# Autodesk Inventor assembly: Assembly1
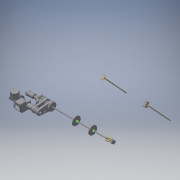
[picture p0: Inventor's stored thumbnail of the model, 180x180]
Saved by Autodesk Inventor 2019 (Build 230136000, 136)
## iProperties
Created: 2019-04-27
Part Number: Assembly1
Document SubType Name: Assembly
Designer: isadmin
Author: isadmin
## Documents named in this file (17)
- C:\Users\isadmin\Documents\Inventor\IS_01\Assembly1.iam
- C:\Users\isadmin\Documents\Inventor\IS_01\670000.ipt
- C:\Users\isadmin\Documents\Inventor\IS_01\CF Insert Flange Support 01.ipt
- C:\Users\isadmin\Documents\Inventor\IS_01\MCF275-FlgMplxr-Cr1A5_(53-321020-A).ipt
- C:\Users\isadmin\Documents\Inventor\IS_01\665501.ipt
- C:\Users\isadmin\Documents\Inventor\IS_01\Rod Central.ipt
- C:\Users\isadmin\Documents\Inventor\IS_01\block.ipt
- C:\Users\isadmin\Documents\Inventor\IS_01\Shield_1.ipt
- C:\Users\isadmin\Documents\Inventor\IS_01\Shield_3.ipt
- C:\Users\isadmin\Documents\Inventor\IS_01\Shutter.ipt
- C:\Users\isadmin\Documents\Inventor\IS_01\ceramic washer.ipt
- C:\Users\isadmin\Documents\Inventor\IS_01\Shielding.ipt
- C:\Users\isadmin\Documents\Inventor\IS_01\alumina_standoff_LSP_ASO00110.ipt
- C:\Users\isadmin\Documents\Inventor\IS_01\Bullet_v5_SiliconeSample.ipt
- C:\Users\isadmin\Documents\Inventor\IS_01\Bullet_v5_SiliconeSample_TopPart.ipt
- C:\Users\isadmin\Documents\Inventor\IS_01\Part8.ipt
- C:\Users\isadmin\Documents\Inventor\IS_01\Part9.ipt
## Components (43 placed, 16 different names)
1. 670000:1 — Insert:1, Insert:4
2. CF Insert Flange Support:1 — Insert:3
3. MCF275-FlgMplxr-Cr1A5_(53-321020-A):1 — Insert:1, Insert:2
4. 665501:1 — Insert:2, Insert:3
5. Rod Central:1 — Insert:4, Insert:5, Insert:7, Insert:8
6. block:1 — Insert:6
7. Shield_1:1 — Mate:32
8. Shield_3:1 — Insert:5
9. Shutter:1
10. ceramic washer:1
11. ceramic washer:2
12. ceramic washer:3
13. ceramic washer:4
14. Shielding:1
15. ceramic washer:5
16. ceramic washer:6
17. ceramic washer:7
18. ceramic washer:8
19. alumina_standoff_LSP_ASO00110:1
20. alumina_standoff_LSP_ASO00110:2
21. alumina_standoff_LSP_ASO00110:3 — Mate:32
22. alumina_standoff_LSP_ASO00110:4
23. Bullet_v5_SiliconeSample:1 — Insert:6
24. Bullet_v5_SiliconeSample_TopPart:1
25. Part8:1 — Insert:7, Insert:9
26. Part8:2 — Insert:8, Insert:10
27. Part9:1 — Insert:9
28. Part9:2 — Insert:10
29. Shield_1:2 — Insert:12, Insert:13
30. block:2 — Insert:12, Insert:13
31. Shutter:2
32. ceramic washer:9
33. ceramic washer:10
34. ceramic washer:11
35. ceramic washer:12
36. Shielding:2
37. ceramic washer:13
38. ceramic washer:14
39. ceramic washer:15
40. ceramic washer:16
41. Bullet_v5_SiliconeSample:2
42. Bullet_v5_SiliconeSample_TopPart:2
43. Shield_1:3
## Relationships (75: Mate 56, Insert 13, Flush 6)
- Insert:1 (-0.254 mm): 670000:1 ↔ MCF275-FlgMplxr-Cr1A5_(53-321020-A):1
- Insert:2 (0.254 mm): MCF275-FlgMplxr-Cr1A5_(53-321020-A):1 ↔ 665501:1
- Insert:3 (0.254 mm): CF Insert Flange Support:1 ↔ 665501:1
- Insert:4: 670000:1 ↔ Rod Central:1
- [Mate]: block:1 ↔ Shield_1:1
- [Flush]: block:1 ↔ Shield_1:1
- [Flush]: block:1 ↔ Shield_1:1
- [Mate]: block:1 ↔ Shutter:1
- [Mate]: block:1 ↔ Shutter:1
- [Mate]: block:1 ↔ Shutter:1
- [Mate]: block:1 ↔ ceramic washer:2
- [Mate]: block:1 ↔ ceramic washer:2
- [Mate]: block:1 ↔ ceramic washer:1
- [Mate]: block:1 ↔ ceramic washer:1
- [Mate]: block:1 ↔ ceramic washer:4
- [Mate]: block:1 ↔ ceramic washer:4
- [Mate]: block:1 ↔ ceramic washer:3
- [Mate]: block:1 ↔ ceramic washer:3
- [Mate]: ceramic washer:1 ↔ Shielding:1
- [Flush]: block:1 ↔ Shielding:1
- [Flush]: block:1 ↔ Shielding:1
- [Mate]: block:1 ↔ ceramic washer:5
- [Mate]: block:1 ↔ ceramic washer:5
- [Mate]: block:1 ↔ ceramic washer:6
- [Mate]: block:1 ↔ ceramic washer:6
- [Mate]: block:1 ↔ ceramic washer:7
- [Mate]: block:1 ↔ ceramic washer:7
- [Mate]: block:1 ↔ ceramic washer:8
- [Mate]: block:1 ↔ ceramic washer:8
- [Mate]: Shield_1:1 ↔ alumina_standoff_LSP_ASO00110:3
- [Mate]: Shield_1:1 ↔ alumina_standoff_LSP_ASO00110:2
- [Mate]: Shield_1:1 ↔ alumina_standoff_LSP_ASO00110:2
- [Mate]: Shield_1:1 ↔ alumina_standoff_LSP_ASO00110:4
- [Mate]: Shield_1:1 ↔ alumina_standoff_LSP_ASO00110:4
- [Mate]: Shield_1:1 ↔ alumina_standoff_LSP_ASO00110:1
- [Mate]: Shield_1:1 ↔ alumina_standoff_LSP_ASO00110:1
- [Mate]: Shield_3:1 ↔ alumina_standoff_LSP_ASO00110:3
- [Mate]: Shield_3:1 ↔ alumina_standoff_LSP_ASO00110:2
- [Mate]: Shield_3:1 ↔ alumina_standoff_LSP_ASO00110:2
- Mate:32: Shield_1:1 ↔ alumina_standoff_LSP_ASO00110:3
- Insert:5: Rod Central:1 ↔ Shield_3:1
- [Mate] (0.0254 mm): Bullet_v5_SiliconeSample:1 ↔ Bullet_v5_SiliconeSample_TopPart:1
- [Mate]: Bullet_v5_SiliconeSample:1 ↔ Bullet_v5_SiliconeSample_TopPart:1
- Insert:6: block:1 ↔ Bullet_v5_SiliconeSample:1
- Insert:7 (-304.8 mm): Rod Central:1 ↔ Part8:1
- Insert:8 (-152.4 mm): Rod Central:1 ↔ Part8:2
- Insert:9 (-12.7 mm): Part8:1 ↔ Part9:1
- Insert:10 (-12.7 mm): Part8:2 ↔ Part9:2
- [Mate]: block:2 ↔ Shutter:2
- [Mate]: block:2 ↔ Shutter:2
- [Mate]: block:2 ↔ Shutter:2
- [Mate]: block:2 ↔ ceramic washer:10
- [Mate]: block:2 ↔ ceramic washer:10
- [Mate]: block:2 ↔ ceramic washer:9
- [Mate]: block:2 ↔ ceramic washer:9
- [Mate]: block:2 ↔ ceramic washer:12
- [Mate]: block:2 ↔ ceramic washer:12
- [Mate]: block:2 ↔ ceramic washer:11
- [Mate]: block:2 ↔ ceramic washer:11
- [Mate]: ceramic washer:9 ↔ Shielding:2
- [Flush]: block:2 ↔ Shielding:2
- [Flush]: block:2 ↔ Shielding:2
- [Mate]: block:2 ↔ ceramic washer:13
- [Mate]: block:2 ↔ ceramic washer:13
- [Mate]: block:2 ↔ ceramic washer:14
- [Mate]: block:2 ↔ ceramic washer:14
- [Mate]: block:2 ↔ ceramic washer:15
- [Mate]: block:2 ↔ ceramic washer:15
- [Mate]: block:2 ↔ ceramic washer:16
- [Mate]: block:2 ↔ ceramic washer:16
- [Mate] (0.0254 mm): Bullet_v5_SiliconeSample:2 ↔ Bullet_v5_SiliconeSample_TopPart:2
- [Mate]: Bullet_v5_SiliconeSample:2 ↔ Bullet_v5_SiliconeSample_TopPart:2
- [Insert]: block:2 ↔ Bullet_v5_SiliconeSample:2
- Insert:12: Shield_1:2 ↔ block:2
- Insert:13: Shield_1:2 ↔ block:2
## Named parameters: d22_d25 = 0 mm, d23_d26 = 0 mm, d24_d35 = 0 mm, d25_d36 = 0 mm, d26_d37 = 0 mm, d27_d38 = 0 mm, d28_d39 = 0 mm, d29_d40 = 0 mm, d30_d41 = 0 mm, d31_d42 = 0 mm, d56_d0 = 0.0254 mm, d57_d1 = 0 mm, d75_d58 = 0 mm, d76_d19 = 0 mm, d77_d22_d25 = 0 mm, d78_d23_d26 = 0 mm, d79_d24_d35 = 0 mm, d80_d25_d36 = 0 mm, d81_d26_d37 = 0 mm, d82_d27_d38 = 0 mm, d83_d28_d39 = 0 mm, d84_d29_d40 = 0 mm, d85_d30_d41 = 0 mm, d86_d31_d42 = 0 mm, d87_d43 = 0 mm, d88_d44 = 0 mm, d89_d45 = 0 mm, d90_d46 = 0 mm, d91_d47 = 0 mm, d92_d48 = 0 mm, d93_d49 = 0 mm, d94_d50 = 0 mm, d95_d51 = 0 mm, d96_d52 = 0 mm, d97_d53 = 0 mm, d98_d56_d0 = 0.0254 mm, d99_d57_d1 = 0 mm
